# Autodesk Inventor assembly: 0002_ASS_Ban_lap_ghep_01
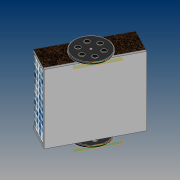
[picture p0: Inventor's stored thumbnail of the model, 180x180]
Saved by Autodesk Inventor 2021 (Build 250183000, 183)
## iProperties
Created: 2024-04-07
Part Number: 0002_ASS_Ban_lap_ghep_01
Document SubType Name: Assembly
Designer: Admin
Author: Admin
## Documents named in this file (5)
- C:\Users\Admin\Desktop\DO_AN_TOT_NGHIEP_2024\Mechanical\Design_in_3D\Version_2\0002_ASS_Ban_lap_ghep_01.iam
- C:\Users\Admin\Desktop\DO_AN_TOT_NGHIEP_2024\Mechanical\Design_in_3D\Version_1\0001_ASS_Hop_so.iam
- C:\Users\Admin\Desktop\DO_AN_TOT_NGHIEP_2024\Mechanical\Design_in_3D\Version_2\01_Tam_de_01.ipt
- C:\Users\Admin\Desktop\DO_AN_TOT_NGHIEP_2024\Mechanical\Design_in_3D\Version_2\02_Tam_hong.ipt
- C:\Users\Admin\Desktop\DO_AN_TOT_NGHIEP_2024\Mechanical\Design_in_3D\Version_2\03_Tam_top_vs_bottom.ipt
## Components (7 placed, 4 different names)
1. 0001_ASS_Hop_so:1 [sub-assembly] — Mate:1, Flush:1, Mate:2, Mate:3, Symmetry:1
2. 0001_ASS_Hop_so:2 [sub-assembly] — Mate:1, Flush:1, Mate:2, Mate:4, Symmetry:1
3. 01_Tam_de_01:1 — Mate:3, Mate:4, Mate:5, Flush:2, Mate:6, Flush:3, Mate:7, Flush:4, Mate:8, Flush:5, Flush:6, Mate:11
4. 02_Tam_hong:1 — Flush:2, Mate:6, Flush:3, Mate:10
5. 03_Tam_top_vs_bottom:1 — Flush:7, Mate:10, Mate:11
6. 02_Tam_hong:2 — Mate:7, Flush:4, Flush:5, Mate:9, Flush:7
7. 03_Tam_top_vs_bottom:2 — Mate:8, Flush:6, Mate:9
## Relationships (19: Mate 11, Flush 7, Symmetry 1)
- Mate:1: 0001_ASS_Hop_so:1 ↔ 0001_ASS_Hop_so:2
- Flush:1: 0001_ASS_Hop_so:1 ↔ 0001_ASS_Hop_so:2
- Mate:2 (10 mm): 0001_ASS_Hop_so:1 ↔ 0001_ASS_Hop_so:2
- Mate:3: 0001_ASS_Hop_so:1 ↔ 01_Tam_de_01:1
- Mate:4: 0001_ASS_Hop_so:2 ↔ 01_Tam_de_01:1
- Symmetry:1: 0001_ASS_Hop_so:1 ↔ 0001_ASS_Hop_so:2
- Mate:5: 01_Tam_de_01:1
- Flush:2: 01_Tam_de_01:1 ↔ 02_Tam_hong:1
- Mate:6: 01_Tam_de_01:1 ↔ 02_Tam_hong:1
- Flush:3: 01_Tam_de_01:1 ↔ 02_Tam_hong:1
- Mate:7: 01_Tam_de_01:1 ↔ 02_Tam_hong:2
- Flush:4: 01_Tam_de_01:1 ↔ 02_Tam_hong:2
- Mate:8: 01_Tam_de_01:1 ↔ 03_Tam_top_vs_bottom:2
- Flush:5: 01_Tam_de_01:1 ↔ 02_Tam_hong:2
- Flush:6: 01_Tam_de_01:1 ↔ 03_Tam_top_vs_bottom:2
- Mate:9: 02_Tam_hong:2 ↔ 03_Tam_top_vs_bottom:2
- Flush:7: 03_Tam_top_vs_bottom:1 ↔ 02_Tam_hong:2
- Mate:10: 02_Tam_hong:1 ↔ 03_Tam_top_vs_bottom:1
- Mate:11: 01_Tam_de_01:1 ↔ 03_Tam_top_vs_bottom:1
